# Autodesk Inventor assembly: LegDemo
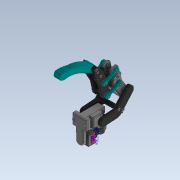
[picture p0: Inventor's stored thumbnail of the model, 180x180]
Saved by Autodesk Inventor 2020 (Build 240168000, 168)
## iProperties
Created: 2019-05-09
Part Number: LegDemo
Document SubType Name: Assembly
Designer: Turing
Author: Turing
## Documents named in this file (35)
- D:\Hexapod Final Fucking Version 2\LegDemoRight.iam
- D:\Hexapod Final Fucking Version 2\Tower Pro MG90S Micro servo.iam
- D:\Hexapod Final Fucking Version 2\Fermur.iam
- D:\Hexapod Final Fucking Version 2\TibiaTop.ipt
- D:\Hexapod Final Fucking Version 2\TCRT5000.ipt
- D:\Hexapod Final Fucking Version 2\Compress Spring1.iam
- D:\Hexapod Final Fucking Version 2\PistonCasingTop.ipt
- D:\Hexapod Final Fucking Version 2\PistonCasingPivot.ipt
- D:\Hexapod Final Fucking Version 2\Tibia Joint.ipt
- D:\Hexapod Final Fucking Version 2\PistonCasingBot.ipt
- D:\Hexapod Final Fucking Version 2\TibiaBot.ipt
- D:\Hexapod Final Fucking Version 2\Fibula.ipt
- D:\Hexapod Final Fucking Version 2\Tarsus.ipt
- D:\Hexapod Final Fucking Version 2\FibulaBot.ipt
- D:\Hexapod Final Fucking Version 2\PatellaBot.ipt
- D:\Hexapod Final Fucking Version 2\PatellaTop.ipt
- D:\Hexapod Final Fucking Version 2\Piston.iam
- D:\Hexapod Final Fucking Version 2\Bolted Connection1.iam
- D:\Hexapod Final Fucking Version 2\Bolted Connection2.iam
- D:\Hexapod Final Fucking Version 2\Bolted Connection3.iam
- D:\Hexapod Final Fucking Version 2\Bolted Connection4.iam
- D:\Hexapod Final Fucking Version 2\Bolted Connection5.iam
- D:\Hexapod Final Fucking Version 2\Bolted Connection6.iam
- D:\Hexapod Final Fucking Version 2\Bolted Connection7.iam
- D:\Hexapod Final Fucking Version 2\Bolted Connection8.iam
- D:\Hexapod Final Fucking Version 2\Bolted Connection9.iam
- D:\Hexapod Final Fucking Version 2\Bolted Connection10.iam
- D:\Hexapod Final Fucking Version 2\Bolted Connection11.iam
- D:\Hexapod Final Fucking Version 2\Bolted Connection12.iam
- D:\Hexapod Final Fucking Version 2\Bearing1.iam
- D:\Hexapod Final Fucking Version 2\Bearing2.iam
- D:\Hexapod Final Fucking Version 2\Bolted Connection13.iam
- D:\Hexapod Final Fucking Version 2\Bolted Connection14.iam
- D:\Hexapod Final Fucking Version 2\Bolted Connection15.iam
- D:\Hexapod Final Fucking Version 2\Bolted Connection16.iam
## Components (39 placed, 18 different names)
1. Tower Pro MG90S Micro servo:1 [sub-assembly] — Rotational:17
2. Tower Pro MG90S Micro servo:2 [sub-assembly] — Rigid:31, Rotational:18, Mate:59, Mate:60
3. Tower Pro MG90S Micro servo:3 [sub-assembly] — Rigid:33, Rotational:19, Mate:61, Mate:62
4. Fermur:1 [sub-assembly] — Rotational:17, Rigid:31, Mate:57, Flush:1, Mate:67, Mate:68, Mate:69, Mate:70, Mate:71, Mate:72
5. TCRT5000:1 — Rigid:26
6. Compress Spring:1 [sub-assembly] — Mate:5, Rigid:35
7. PistonCasingTop:1 — Rigid:24
8. PistonCasingBot:1 — Rigid:24, Rigid:25, Slider:1, Mate:65, Mate:66
9. PistonCasingPivot:1 — Rigid:25, Rigid:26, Mate:53, Mate:63, Mate:64
10. FibulaBot:1 — Rigid:37, Rotational:24, Angle:14
11. Fibula:2 — Rigid:36, Mate:51, Mate:52, Mate:55, Mate:56
12. Piston:1 [sub-assembly] — Mate:5, Rigid:35, Slider:1, Mate:54
13. Tarsus:1 — Rigid:36, Rigid:37
14. PatellaBot:1 — Rotational:18, Rigid:32, Rigid:33
15. PatellaTop:1 — Rigid:32, Mate:37, Mate:38, Mate:58, Flush:2
16. TibiaTop:2 — Rigid:34, Rotational:22, Rotational:23, Mate:39, Mate:40, Mate:49, Mate:50
17. TibiaBot:1 — Rotational:19, Rigid:34, Rotational:20, Rotational:21, Angle:14
18. Tibia Joint:1 — Rotational:21, Angle:11, Mate:47, Mate:48
19. Tibia Joint:2 — Rotational:23, Angle:12, Mate:41, Mate:42
20. Tibia Joint:3 — Rotational:20, Angle:11, Angle:12, Angle:13, Rotational:24, Mate:43, Mate:44
21. Tibia Joint:4 — Rotational:22, Angle:13, Mate:45, Mate:46
22. Leg Bolted Connection:1 [sub-assembly] — Mate:69, Mate:70
23. Leg Bolted Connection:2 [sub-assembly] — Mate:71, Mate:72
24. Leg Bolted Connection:3 [sub-assembly] — Mate:67, Mate:68
25. Leg Bolted Connection:4 [sub-assembly] — Mate:37, Mate:38
26. Leg Bolted Connection:5 [sub-assembly] — Mate:39, Mate:40
27. Leg Bolted Connection:6 [sub-assembly] — Mate:41, Mate:42
28. Leg Bolted Connection:7 [sub-assembly] — Mate:43, Mate:44
29. Leg Bolted Connection:8 [sub-assembly] — Mate:45, Mate:46
30. Leg Bolted Connection:9 [sub-assembly] — Mate:47, Mate:48
31. Leg Bolted Connection:10 [sub-assembly] — Mate:49, Mate:50, Mate:53
32. Leg Bolted Connection:11 [sub-assembly] — Mate:51, Mate:52, Mate:54
33. Leg Bolted Connection:12 [sub-assembly] — Mate:55, Mate:56
34. Leg Bearing:1 [sub-assembly] — Mate:57, Flush:1
35. Leg Bearing:2 [sub-assembly] — Mate:58, Flush:2
36. Leg Bolted Connection:13 [sub-assembly] — Mate:59, Mate:60
37. Leg Bolted Connection:14 [sub-assembly] — Mate:61, Mate:62
38. Leg Bolted Connection:15 [sub-assembly] — Mate:63, Mate:64
39. Leg Bolted Connection:16 [sub-assembly] — Mate:65, Mate:66
## Relationships (62: Mate 37, WeldJoint 10, RevoluteJoint 8, Angle 4, Flush 2, TranslationJoint 1)
- Rigid:24 [WeldJoint]: PistonCasingTop:1 ↔ PistonCasingBot:1
- Rigid:25 [WeldJoint]: PistonCasingBot:1 ↔ PistonCasingPivot:1
- Rigid:26 [WeldJoint]: TCRT5000:1 ↔ PistonCasingPivot:1
- Rotational:17 [RevoluteJoint]: Tower Pro MG90S Micro servo:1 ↔ Fermur:1
- Rigid:31 [WeldJoint]: Tower Pro MG90S Micro servo:2 ↔ Fermur:1
- Rotational:18 [RevoluteJoint]: Tower Pro MG90S Micro servo:2 ↔ PatellaBot:1
- Rigid:32 [WeldJoint]: PatellaBot:1 ↔ PatellaTop:1
- Rigid:33 [WeldJoint]: Tower Pro MG90S Micro servo:3 ↔ PatellaBot:1
- Rotational:19 [RevoluteJoint]: Tower Pro MG90S Micro servo:3 ↔ TibiaBot:1
- Rigid:34 [WeldJoint]: TibiaTop:2 ↔ TibiaBot:1
- Rotational:20 [RevoluteJoint]: TibiaBot:1 ↔ Tibia Joint:3
- Rotational:21 [RevoluteJoint]: TibiaBot:1 ↔ Tibia Joint:1
- Angle:11 (0 deg): Tibia Joint:1 ↔ Tibia Joint:3
- Rotational:22 [RevoluteJoint]: TibiaTop:2 ↔ Tibia Joint:4
- Rotational:23 [RevoluteJoint]: TibiaTop:2 ↔ Tibia Joint:2
- Angle:12 (180 deg): Tibia Joint:2 ↔ Tibia Joint:3
- Angle:13 (0 deg): Tibia Joint:3 ↔ Tibia Joint:4
- Mate:5: Compress Spring:1 ↔ Piston:1
- Rigid:35 [WeldJoint]: Compress Spring:1 ↔ Piston:1
- Rigid:36 [WeldJoint]: Fibula:2 ↔ Tarsus:1
- Rigid:37 [WeldJoint]: FibulaBot:1 ↔ Tarsus:1
- Rotational:24 [RevoluteJoint]: FibulaBot:1 ↔ Tibia Joint:3
- Angle:14 (0 deg): FibulaBot:1 ↔ TibiaBot:1
- Slider:1 [TranslationJoint]: PistonCasingBot:1 ↔ Piston:1
- Mate:37: PatellaTop:1 ↔ Leg Bolted Connection:4
- Mate:38: PatellaTop:1 ↔ Leg Bolted Connection:4
- Mate:39: TibiaTop:2 ↔ Leg Bolted Connection:5
- Mate:40: TibiaTop:2 ↔ Leg Bolted Connection:5
- Mate:41: Tibia Joint:2 ↔ Leg Bolted Connection:6
- Mate:42: Tibia Joint:2 ↔ Leg Bolted Connection:6
- Mate:43: Tibia Joint:3 ↔ Leg Bolted Connection:7
- Mate:44: Tibia Joint:3 ↔ Leg Bolted Connection:7
- Mate:45: Tibia Joint:4 ↔ Leg Bolted Connection:8
- Mate:46: Tibia Joint:4 ↔ Leg Bolted Connection:8
- Mate:47: Tibia Joint:1 ↔ Leg Bolted Connection:9
- Mate:48: Tibia Joint:1 ↔ Leg Bolted Connection:9
- Mate:49: TibiaTop:2 ↔ Leg Bolted Connection:10
- Mate:50: TibiaTop:2 ↔ Leg Bolted Connection:10
- Mate:51: Fibula:2 ↔ Leg Bolted Connection:11
- Mate:52: Fibula:2 ↔ Leg Bolted Connection:11
- Mate:53: PistonCasingPivot:1 ↔ Leg Bolted Connection:10
- Mate:54: Piston:1 ↔ Leg Bolted Connection:11
- Mate:55: Fibula:2 ↔ Leg Bolted Connection:12
- Mate:56: Fibula:2 ↔ Leg Bolted Connection:12
- Mate:57: Fermur:1 ↔ Leg Bearing:1
- Flush:1: Fermur:1 ↔ Leg Bearing:1
- Mate:58: PatellaTop:1 ↔ Leg Bearing:2
- Flush:2: PatellaTop:1 ↔ Leg Bearing:2
- Mate:59: Tower Pro MG90S Micro servo:2 ↔ Leg Bolted Connection:13
- Mate:60: Tower Pro MG90S Micro servo:2 ↔ Leg Bolted Connection:13
- Mate:61: Tower Pro MG90S Micro servo:3 ↔ Leg Bolted Connection:14
- Mate:62: Tower Pro MG90S Micro servo:3 ↔ Leg Bolted Connection:14
- Mate:63: PistonCasingPivot:1 ↔ Leg Bolted Connection:15
- Mate:64: PistonCasingPivot:1 ↔ Leg Bolted Connection:15
- Mate:65: PistonCasingBot:1 ↔ Leg Bolted Connection:16
- Mate:66: PistonCasingBot:1 ↔ Leg Bolted Connection:16
- Mate:67: Fermur:1 ↔ Leg Bolted Connection:3
- Mate:68: Fermur:1 ↔ Leg Bolted Connection:3
- Mate:69: Fermur:1 ↔ Leg Bolted Connection:1
- Mate:70: Fermur:1 ↔ Leg Bolted Connection:1
- Mate:71: Fermur:1 ↔ Leg Bolted Connection:2
- Mate:72: Fermur:1 ↔ Leg Bolted Connection:2
